# Autodesk Inventor assembly: Batteria e connettore
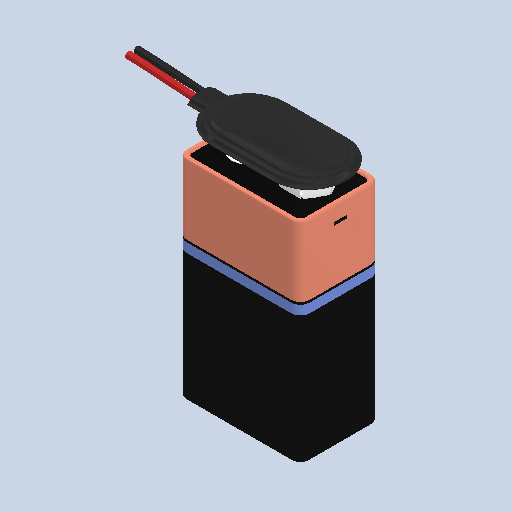
[picture p0: Inventor's stored thumbnail of the model, 512x512]
Saved by Autodesk Inventor 2023 (Build 270158000, 158)
## iProperties
Created: 2022-12-31
Part Number: Batteria e connettore
Document SubType Name: Assembly
Designer: Gabriele
Author: Gabriele
## Documents named in this file (3)
- C:\Users\Gabriele\Desktop\Progetto Lab\AY2223_I_Project-2\3D\Case\Batteria e connettore.iam
- C:\Users\Gabriele\Desktop\Progetto Lab\AY2223_I_Project-2\3D\Case\9V Battery.ipt
- C:\Users\Gabriele\Desktop\Progetto Lab\AY2223_I_Project-2\3D\Case\9V Battery Clip Connector.ipt
## Components (2 placed, 2 different names)
1. 9V Battery:1 — Coincidente:1, Allineato:1, Allineato:2
2. 9V Battery Clip Connector:1 — Coincidente:1, Allineato:1, Allineato:2
## Relationships (3: Flush 2, Mate 1)
- Coincidente:1 [Mate] (4 mm): 9V Battery:1 ↔ 9V Battery Clip Connector:1
- Allineato:1 [Flush] (-3.5 mm): 9V Battery:1 ↔ 9V Battery Clip Connector:1
- Allineato:2 [Flush] (0.6 mm): 9V Battery:1 ↔ 9V Battery Clip Connector:1
